# Autodesk Inventor assembly: Sensor_Box_Assembly.ipt
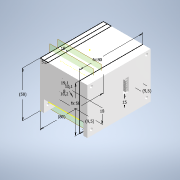
[picture p0: Inventor's stored thumbnail of the model, 180x180]
Saved by Autodesk Inventor 2022 (Build 260153000, 153)
## iProperties
Created: 2022-10-05
Part Number: Sensor_Box_Assembly.ipt
Document SubType Name: Assembly
Designer: alexw
Mass: 258.974 g
Surface Area: 609.263 cm^2
Volume: 185.802 cm^3
Author: alexw
## Documents named in this file (9)
- C:\Users\AEWALDER\Documents\Inventor\03_CurrentProjects\MasterThesis\PSM_V1_Rillenkugellager\Sensor_Box_Assembly.ipt.iam
- C:\Users\AEWALDER\Documents\Inventor\03_CurrentProjects\MasterThesis\PSM_V1_Rillenkugellager\daVinci_Head_Sensorpart.ipt
- C:\Users\AEWALDER\Documents\Inventor\03_CurrentProjects\MasterThesis\PSM_V1_Rillenkugellager\Sensor_Box_Deckel.ipt
- C:\Users\AEWALDER\Documents\Inventor\03_CurrentProjects\MasterThesis\PSM_V1_Rillenkugellager\AVAGO_HEDS_5540_A1.ipt
- C:\Users\AEWALDER\Documents\Inventor\03_CurrentProjects\MasterThesis\PSM_V1_Rillenkugellager\Maschinenbauteil\WBB1-8705\SKF_WBB1-8705.iam
- C:\Users\AEWALDER\Documents\Inventor\03_CurrentProjects\MasterThesis\PSM_V1_Rillenkugellager\Abdeckung_Sensorkopfh.ipt
- C:\Users\AEWALDER\Documents\Inventor\03_CurrentProjects\MasterThesis\PSM_V1_Rillenkugellager\Maschinenbauteil\623-2RS1\SKF_623-2RS1.iam
- C:\Users\AEWALDER\Documents\Inventor\03_CurrentProjects\MasterThesis\PSM_V1_Rillenkugellager\SensorKopf_Encoder_Welle.ipt
- C:\Users\AEWALDER\Documents\Inventor\03_CurrentProjects\MasterThesis\PSM_V1_Rillenkugellager\Riemenscheibe.ipt
## Components (8 placed, 8 different names)
1. daVinci_Head_Sensorpart:1 — Fluchtend:1, Fluchtend:2, Fluchtend:3, Passend:3, Passend:4, Passend:5, Fluchtend:6, Mate:6, Mate:7, Mate:8, Mate:11, Flush:8, Mate:12, Mate:13, Mate:14, Mate:15, Mate:19
2. Sensor_Box_Deckel:1 — Passend:3, Passend:4, Passend:5
3. AVAGO_HEDS_5540_A1:1 — Mate:6, Mate:7, Mate:8
4. SKF_623-2RS1:1 [sub-assembly] — Mate:14, Mate:15, Mate:16, Mate:17
5. SKF_WBB1-8705:1 [sub-assembly] — Mate:11, Flush:8
6. Abdeckung_Sensorkopfh:1 — Mate:12, Mate:13
7. SensorKopf_Encoder_Welle:1 — Mate:16, Mate:17, Mate:18
8. Riemenscheibe:1 — Mate:18, Mate:19
## Relationships (21: Mate 15, Flush 6)
- Fluchtend:1 [Flush]: daVinci_Head_Sensorpart:1
- Fluchtend:2 [Flush]: daVinci_Head_Sensorpart:1
- Fluchtend:3 [Flush]: daVinci_Head_Sensorpart:1
- Passend:3 [Mate]: daVinci_Head_Sensorpart:1 ↔ Sensor_Box_Deckel:1
- Passend:4 [Mate]: daVinci_Head_Sensorpart:1 ↔ Sensor_Box_Deckel:1
- Passend:5 [Mate]: daVinci_Head_Sensorpart:1 ↔ Sensor_Box_Deckel:1
- Fluchtend:6 [Flush] (5.5 mm): daVinci_Head_Sensorpart:1
- Fluchtend:7 [Flush] (10 mm)
- Mate:6: daVinci_Head_Sensorpart:1 ↔ AVAGO_HEDS_5540_A1:1
- Mate:7: daVinci_Head_Sensorpart:1 ↔ AVAGO_HEDS_5540_A1:1
- Mate:8: daVinci_Head_Sensorpart:1 ↔ AVAGO_HEDS_5540_A1:1
- Mate:11: daVinci_Head_Sensorpart:1 ↔ SKF_WBB1-8705:1
- Flush:8: daVinci_Head_Sensorpart:1 ↔ SKF_WBB1-8705:1
- Mate:12: daVinci_Head_Sensorpart:1 ↔ Abdeckung_Sensorkopfh:1
- Mate:13: daVinci_Head_Sensorpart:1 ↔ Abdeckung_Sensorkopfh:1
- Mate:14: daVinci_Head_Sensorpart:1 ↔ SKF_623-2RS1:1
- Mate:15: daVinci_Head_Sensorpart:1 ↔ SKF_623-2RS1:1
- Mate:16: SKF_623-2RS1:1 ↔ SensorKopf_Encoder_Welle:1
- Mate:17: SKF_623-2RS1:1 ↔ SensorKopf_Encoder_Welle:1
- Mate:18: SensorKopf_Encoder_Welle:1 ↔ Riemenscheibe:1
- Mate:19 (6.25 mm): daVinci_Head_Sensorpart:1 ↔ Riemenscheibe:1
